# Autodesk Inventor assembly: 機体下部
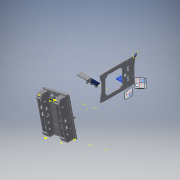
[picture p0: Inventor's stored thumbnail of the model, 180x180]
Saved by Autodesk Inventor 2018 (Build 220112000, 112)
## iProperties
Created: 2018-08-16
Part Number: 機体下部
Material: 一般
Document SubType Name: Assembly
Designer: shun2
Author: shun2
## Documents named in this file (12)
- C:\Users\shun2\OneDrive\おそらく最新版(2018.7.31)\機体下部.iam
- C:\Users\shun2\OneDrive\おそらく最新版(2018.7.31)\ギアボックス\ギアボックス片側.iam
- C:\Users\shun2\OneDrive\おそらく最新版(2018.7.31)\1枚目\一枚目.ipt
- C:\Users\shun2\OneDrive\おそらく最新版(2018.7.31)\2枚目\2枚目.ipt
- C:\Users\shun2\OneDrive\おそらく最新版(2018.7.31)\モタドラ.ipt
- C:\Users\shun2\OneDrive\おそらく最新版(2018.7.31)\基板保護2018.8.7.ipt
- C:\Users\shun2\OneDrive\おそらく最新版(2018.7.31)\ステッピング固定具.ipt
- C:\Users\shun2\OneDrive\おそらく最新版(2018.7.31)\Color.ipt
- C:\Users\shun2\OneDrive\おそらく最新版(2018.7.31)\レスキューキット投下機構.ipt
- C:\Users\shun2\OneDrive\おそらく最新版(2018.7.31)\3枚目\3枚目v2.ipt
- C:\Users\shun2\OneDrive\おそらく最新版(2018.7.31)\PingCover.ipt
- C:\Users\shun2\OneDrive\おそらく最新版(2018.7.31)\ping.ipt
## Components (13 placed, 11 different names)
1. ギアボックス片側:1 [sub-assembly] — メイト:17, メイト:18, メイト:21, メイト:22, メイト:41, メイト:57
2. ギアボックス片側:2 [sub-assembly] — メイト:19, メイト:20, メイト:21, メイト:22, メイト:42, メイト:57, メイト:58, フラッシュ:1
3. 一枚目:1 — メイト:1, メイト:3, メイト:5, メイト:6, メイト:10, メイト:11, メイト:14, メイト:15, メイト:16, メイト:30, メイト:31, メイト:32, メイト:33, メイト:36, メイト:37, メイト:38, メイト:39, メイト:41, メイト:42, メイト:56, メイト:58, フラッシュ:1
4. 2枚目:1 — メイト:2, メイト:4, メイト:25, メイト:26, メイト:40, メイト:47, メイト:48, メイト:49, メイト:50, メイト:55, メイト:63, メイト:64, メイト:65, メイト:66, メイト:76, メイト:77, メイト:78, メイト:79
5. モタドラ:1 — メイト:12, メイト:13, メイト:14, メイト:15, メイト:16, メイト:56
6. 基板保護2018.8.7:1 — メイト:28, メイト:29, メイト:30, メイト:31, メイト:39, メイト:40
7. ステッピング固定具:1 — メイト:43, メイト:44, メイト:45, メイト:46, メイト:55, メイト:59, メイト:72, メイト:75, メイト:76, メイト:77, メイト:78
8. Color:1 — メイト:34, メイト:35, メイト:36, メイト:37, メイト:38
9. レスキューキット投下機構:1 — メイト:60, メイト:71, メイト:74, メイト:75, メイト:79
10. 3枚目v2:1 — メイト:80, メイト:81, メイト:82
11. PingCover:1 — メイト:80, メイト:81, メイト:82
12. ping:1
13. PingCover:2
## Relationships (67: Mate 66, Flush 1)
- メイト:1 [Mate]: 一枚目:1
- メイト:2 [Mate]: 2枚目:1
- メイト:3 [Mate]: 一枚目:1
- メイト:4 [Mate]: 2枚目:1
- メイト:5 [Mate]: 一枚目:1
- メイト:6 [Mate]: 一枚目:1
- メイト:10 [Mate]: 一枚目:1
- メイト:11 [Mate]: 一枚目:1
- メイト:12 [Mate]: モタドラ:1
- メイト:13 [Mate]: モタドラ:1
- メイト:14 [Mate]: 一枚目:1 ↔ モタドラ:1
- メイト:15 [Mate]: 一枚目:1 ↔ モタドラ:1
- メイト:16 [Mate]: 一枚目:1 ↔ モタドラ:1
- メイト:17 [Mate]: ギアボックス片側:1
- メイト:18 [Mate]: ギアボックス片側:1
- メイト:19 [Mate]: ギアボックス片側:2
- メイト:20 [Mate]: ギアボックス片側:2
- メイト:21 [Mate]: ギアボックス片側:1 ↔ ギアボックス片側:2
- メイト:22 [Mate]: ギアボックス片側:1 ↔ ギアボックス片側:2
- メイト:25 [Mate]: 2枚目:1
- メイト:26 [Mate]: 2枚目:1
- メイト:27 [Mate]
- メイト:28 [Mate]: 基板保護2018.8.7:1
- メイト:29 [Mate]: 基板保護2018.8.7:1
- メイト:30 [Mate]: 一枚目:1 ↔ 基板保護2018.8.7:1
- メイト:31 [Mate]: 一枚目:1 ↔ 基板保護2018.8.7:1
- メイト:32 [Mate]: 一枚目:1
- メイト:33 [Mate]: 一枚目:1
- メイト:34 [Mate]: Color:1
- メイト:35 [Mate]: Color:1
- メイト:36 [Mate]: 一枚目:1 ↔ Color:1
- メイト:37 [Mate]: 一枚目:1 ↔ Color:1
- メイト:38 [Mate] (3.846 mm): 一枚目:1 ↔ Color:1
- メイト:39 [Mate] (0.559 mm): 一枚目:1 ↔ 基板保護2018.8.7:1
- メイト:40 [Mate] (0.576 mm): 2枚目:1 ↔ 基板保護2018.8.7:1
- メイト:41 [Mate] (2.5 mm): ギアボックス片側:1 ↔ 一枚目:1
- メイト:42 [Mate] (2.5 mm): ギアボックス片側:2 ↔ 一枚目:1
- メイト:43 [Mate]: ステッピング固定具:1
- メイト:44 [Mate]: ステッピング固定具:1
- メイト:45 [Mate]: ステッピング固定具:1
- メイト:46 [Mate]: ステッピング固定具:1
- メイト:47 [Mate]: 2枚目:1
- メイト:48 [Mate]: 2枚目:1
- メイト:49 [Mate]: 2枚目:1
- メイト:50 [Mate]: 2枚目:1
- メイト:55 [Mate] (15 mm): 2枚目:1 ↔ ステッピング固定具:1
- メイト:56 [Mate] (8 mm): 一枚目:1 ↔ モタドラ:1
- メイト:57 [Mate] (73.5 mm): ギアボックス片側:1 ↔ ギアボックス片側:2
- メイト:58 [Mate] (-129.5 mm): ギアボックス片側:2 ↔ 一枚目:1
- フラッシュ:1 [Flush] (-1.8 mm): ギアボックス片側:2 ↔ 一枚目:1
- メイト:59 [Mate]: ステッピング固定具:1
- メイト:60 [Mate]: レスキューキット投下機構:1
- メイト:63 [Mate]: 2枚目:1
- メイト:64 [Mate]: 2枚目:1
- メイト:65 [Mate]: 2枚目:1
- メイト:66 [Mate]: 2枚目:1
- メイト:71 [Mate]: レスキューキット投下機構:1
- メイト:72 [Mate]: ステッピング固定具:1
- メイト:74 [Mate]: レスキューキット投下機構:1
- メイト:75 [Mate]: ステッピング固定具:1 ↔ レスキューキット投下機構:1
- メイト:76 [Mate]: 2枚目:1 ↔ ステッピング固定具:1
- メイト:77 [Mate]: 2枚目:1 ↔ ステッピング固定具:1
- メイト:78 [Mate] (13 mm): 2枚目:1 ↔ ステッピング固定具:1
- メイト:79 [Mate] (2 mm): 2枚目:1 ↔ レスキューキット投下機構:1
- メイト:80 [Mate]: 3枚目v2:1 ↔ PingCover:1
- メイト:81 [Mate]: 3枚目v2:1 ↔ PingCover:1
- メイト:82 [Mate]: 3枚目v2:1 ↔ PingCover:1
